# Autodesk Inventor assembly: A_Airbert
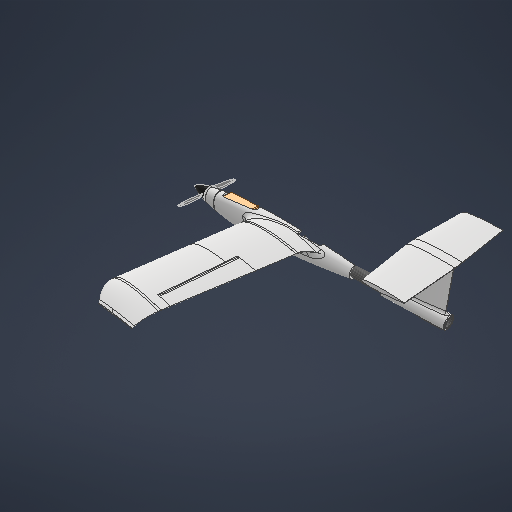
[picture p0: Inventor's stored thumbnail of the model, 512x512]
Saved by Autodesk Inventor 2026 (Build 300175000, 175)
## iProperties
Created: 2025-08-22
Part Number: A_Airbert
Document SubType Name: Assembly
Designer: FAL
Mass: 1109.32 g
Surface Area: 4436.66 cm^2
Volume: 1446.14 cm^3
Density: 0.767087 g/cm^3
Author: FAL
## Documents named in this file (23)
- C:\Users\FAL\Projekte\Git\AIR-BERT\CAD\A_Airbert.iam
- C:\Users\FAL\Projekte\Git\AIR-BERT\CAD\P_Fuselage.ipt
- C:\Users\FAL\Projekte\Git\AIR-BERT\CAD\P_Carbon_Pipe_Back.ipt
- C:\Users\FAL\Projekte\Git\AIR-BERT\CAD\extern\P_AP-PR-006_6-2_LH.ipt
- C:\Users\FAL\Projekte\Git\AIR-BERT\CAD\P_aft_V.ipt
- C:\Users\FAL\Projekte\Git\AIR-BERT\CAD\extern\P_Akku_Dummy.ipt
- C:\Users\FAL\Projekte\Git\AIR-BERT\CAD\P_aft_T.ipt
- P_aft_T.ipt
- C:\Users\FAL\Projekte\Git\AIR-BERT\CAD\extern\P_BLDC_2200KV.ipt
- C:\Users\FAL\Projekte\Git\AIR-BERT\CAD\extern\P_Receiver_Radiolink.ipt
- C:\Users\FAL\Projekte\Git\AIR-BERT\CAD\extern\P_ESC_40A.ipt
- C:\Users\FAL\Projekte\Git\AIR-BERT\CAD\P_aft_X.ipt
- P_aft_X.ipt
- C:\Users\FAL\Projekte\Git\AIR-BERT\CAD\P_MotorNose.ipt
- C:\Users\FAL\Projekte\Git\AIR-BERT\CAD\P_Fuselage_cuts.ipt
- P_Fuselage_Cuts.ipt
- C:\Users\FAL\Projekte\Git\AIR-BERT\CAD\P_Fuselage_Body.ipt
- C:\Users\FAL\Projekte\Git\AIR-BERT\CAD\P_Fuselage_Nose.ipt
- C:\Users\FAL\Projekte\Git\AIR-BERT\CAD\extern\P_Servo_SIMPROP.ipt
- C:\Users\FAL\Projekte\Git\AIR-BERT\CAD\extern\P_Wing_inner.ipt
- C:\Users\FAL\Projekte\Git\AIR-BERT\CAD\extern\P_Wing_mid.ipt
- C:\Users\FAL\Projekte\Git\AIR-BERT\CAD\extern\P_Wing_winglet.ipt
- C:\Users\FAL\Projekte\Git\AIR-BERT\CAD\extern\P_Wing_aileron.ipt
## Components (20 placed, 19 different names)
1. P_Servo_SIMPROP:2
2. P_Servo_SIMPROP:1
3. P_AP-PR-006_6-2_LH:1 — Passend:14
4. P_MotorNose:1 — Passend:22
5. P_Akku_Dummy:1 — Passend:7
6. P_ESC_40A:1
7. P_Receiver_Radiolink:1
8. P_BLDC_2200KV:1 — Passend:12
9. P_Carbon_Pipe_Back:1 — Passend:6, Fluchtend:9, Passend:10, Fluchtend:10, Passend:15, Passend:16, Passend:21, Passend:28
10. P_aft_V:1 — Passend:6, Fluchtend:8, Fluchtend:9
11. P_aft_T:1 — Passend:9, Passend:10, Fluchtend:10
12. P_aft_X:1 — Passend:18, Passend:21, Passend:28
13. P_Fuselage_Body:1 — Fluchtend:28, Fluchtend:29, Fluchtend:30
14. P_Fuselage_Nose:1 — Fluchtend:32, Fluchtend:42, Fluchtend:43
15. P_Fuselage:2 — Fluchtend:11, Fluchtend:12, Fluchtend:13, Passend:15, Passend:16
16. P_Fuselage_Cuts:1 — Fluchtend:14, Fluchtend:15, Fluchtend:16
17. P_Wing_aileron:1 — Fluchtend:44, Fluchtend:45, Fluchtend:46
18. P_Wing_inner:1 — Fluchtend:33, Fluchtend:34, Fluchtend:35
19. P_Wing_mid:1 — Fluchtend:36, Fluchtend:37, Fluchtend:38
20. P_Wing_winglet:1 — Fluchtend:39, Fluchtend:40, Fluchtend:41
## Relationships (39: Flush 27, Mate 12)
- Passend:6 [Mate]: P_Carbon_Pipe_Back:1 ↔ P_aft_V:1
- Fluchtend:8 [Flush]: P_aft_V:1
- Passend:7 [Mate]: P_Akku_Dummy:1
- Fluchtend:9 [Flush]: P_Carbon_Pipe_Back:1 ↔ P_aft_V:1
- Passend:9 [Mate]: P_aft_T:1
- Passend:10 [Mate]: P_Carbon_Pipe_Back:1 ↔ P_aft_T:1
- Fluchtend:10 [Flush]: P_Carbon_Pipe_Back:1 ↔ P_aft_T:1
- Passend:12 [Mate]: P_BLDC_2200KV:1
- Passend:14 [Mate]: P_AP-PR-006_6-2_LH:1
- Fluchtend:11 [Flush]: P_Fuselage:2
- Fluchtend:12 [Flush]: P_Fuselage:2
- Fluchtend:13 [Flush]: P_Fuselage:2
- Passend:15 [Mate]: P_Carbon_Pipe_Back:1 ↔ P_Fuselage:2
- Passend:16 [Mate] (-60 mm): P_Carbon_Pipe_Back:1 ↔ P_Fuselage:2
- Passend:18 [Mate]: P_aft_X:1
- Passend:21 [Mate]: P_Carbon_Pipe_Back:1 ↔ P_aft_X:1
- Passend:22 [Mate]: P_MotorNose:1
- Fluchtend:14 [Flush]: P_Fuselage_Cuts:1
- Fluchtend:15 [Flush]: P_Fuselage_Cuts:1
- Fluchtend:16 [Flush]: P_Fuselage_Cuts:1
- Fluchtend:28 [Flush]: P_Fuselage_Body:1
- Fluchtend:29 [Flush]: P_Fuselage_Body:1
- Fluchtend:30 [Flush]: P_Fuselage_Body:1
- Fluchtend:32 [Flush]: P_Fuselage_Nose:1
- Fluchtend:42 [Flush]: P_Fuselage_Nose:1
- Fluchtend:43 [Flush]: P_Fuselage_Nose:1
- Passend:28 [Mate]: P_Carbon_Pipe_Back:1 ↔ P_aft_X:1
- Fluchtend:33 [Flush]: P_Wing_inner:1
- Fluchtend:34 [Flush]: P_Wing_inner:1
- Fluchtend:35 [Flush]: P_Wing_inner:1
- Fluchtend:36 [Flush]: P_Wing_mid:1
- Fluchtend:37 [Flush]: P_Wing_mid:1
- Fluchtend:38 [Flush]: P_Wing_mid:1
- Fluchtend:39 [Flush]: P_Wing_winglet:1
- Fluchtend:40 [Flush]: P_Wing_winglet:1
- Fluchtend:41 [Flush]: P_Wing_winglet:1
- Fluchtend:44 [Flush]: P_Wing_aileron:1
- Fluchtend:45 [Flush]: P_Wing_aileron:1
- Fluchtend:46 [Flush]: P_Wing_aileron:1
